# Autodesk Inventor assembly: Assembly1
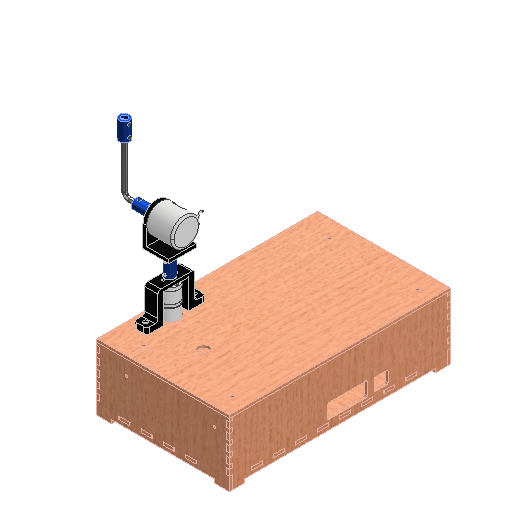
[picture p0: Inventor's stored thumbnail of the model, 512x512]
Saved by Autodesk Inventor 2025.2 (Build 292293000, 293)
## iProperties
Created: 2025-12-07
Part Number: Assembly1
Document SubType Name: Assembly
Designer: hazem
Author: hazem
## Documents named in this file (16)
- D:\Senior 2 MCT\Fall 2025\Hybrid Control\Project\CAD\Workspaces\Workspace\Assembly1.iam
- D:\Senior 2 MCT\Fall 2025\Hybrid Control\Project\CAD\Workspaces\Workspace\Encoder_Default_sldprt.ipt
- D:\Senior 2 MCT\Fall 2025\Hybrid Control\Project\CAD\Workspaces\Workspace\encoderBracketInventor.stp_Default_sldprt.ipt
- D:\Senior 2 MCT\Fall 2025\Hybrid Control\Project\CAD\Workspaces\Workspace\Motor_Default_sldprt.ipt
- D:\Senior 2 MCT\Fall 2025\Hybrid Control\Project\CAD\Workspaces\Workspace\Upper.ipt
- D:\Senior 2 MCT\Fall 2025\Hybrid Control\Project\CAD\Workspaces\Workspace\ground.ipt
- D:\Senior 2 MCT\Fall 2025\Hybrid Control\Project\CAD\Workspaces\Workspace\side.ipt
- D:\Senior 2 MCT\Fall 2025\Hybrid Control\Project\CAD\Workspaces\Workspace\Allen 5 mm.ipt
- D:\Senior 2 MCT\Fall 2025\Hybrid Control\Project\CAD\Workspaces\Workspace\Shaft Coupler 8-5mm.ipt
- D:\Senior 2 MCT\Fall 2025\Hybrid Control\Project\CAD\Workspaces\Workspace\side2.ipt
- D:\Senior 2 MCT\Fall 2025\Hybrid Control\Project\CAD\Workspaces\Workspace\back.ipt
- D:\Senior 2 MCT\Fall 2025\Hybrid Control\Project\CAD\Workspaces\Workspace\Front.ipt
- D:\Senior 2 MCT\Fall 2025\Hybrid Control\Project\CAD\Workspaces\Workspace\L connection.ipt
- D:\Senior 2 MCT\Fall 2025\Hybrid Control\Project\CAD\Workspaces\Workspace\Motor _Fixation.ipt
- D:\Senior 2 MCT\Fall 2025\Hybrid Control\Project\CAD\Workspaces\Workspace\AcoplamentoRigido8x8.ipt
- D:\Senior 2 MCT\Fall 2025\Hybrid Control\Project\CAD\Workspaces\Workspace\Motor Sleeve 0.2.ipt
## Components (22 placed, 15 different names)
1. ground:1 — Mate:31, Flush:12, Flush:13, Mate:39
2. Upper:1 — Flush:7, Flush:9, Flush:10, Mate:46, Mate:49, Mate:50, Mate:53
3. side:1 — Flush:7, Flush:9, Mate:31, Flush:12, Flush:13, Flush:17, Flush:20, Mate:44, Mate:45, Mate:47, Mate:48
4. side2:1 — Flush:10, Flush:18, Flush:21, Mate:51, Mate:52, Mate:54, Mate:55, Flush:22, Mate:56
5. Shaft Coupler 8-5mm:1 — Mate:35, Flush:14
6. Allen 5 mm:1 — Mate:35, Flush:14
7. back:1 — Mate:39, Flush:17, Flush:18, Mate:56, Mate:57
8. Front:1 — Flush:20, Flush:21, Flush:22
9. L connection:1 — Mate:47, Mate:48, Mate:49
10. L connection:2 — Mate:44, Mate:45, Mate:46, Mate:58
11. L connection:3 — Mate:50, Mate:51, Mate:52
12. L connection:4 — Mate:53, Mate:54, Mate:55, Mate:59
13. Motor _Fixation:1 — Mate:61, Mate:62, Mate:63, Mate:64
14. Motor_Default_sldprt:1 — Mate:60, Mate:61, Mate:62, Mate:65, Flush:23
15. Upper:2 — Mate:57, Mate:58, Mate:59, Mate:60, Mate:63, Mate:64
16. AcoplamentoRigido8x8:1 — Mate:66, Flush:24, Mate:67, Mate:68
17. Motor Sleeve 0.2:1 — Mate:65, Flush:23, Mate:66, Flush:24
18. Encoder_Default_sldprt:1 — Mate:69, Mate:70, Mate:71, Mate:72, Mate:75, Mate:76
19. encoderBracketInventor.stp_Default_sldprt:1 — Mate:67, Mate:68, Mate:69, Mate:70, Mate:71, Mate:72
20. Shaft Coupler 8-5mm:2 — Mate:74, Flush:26, Mate:75, Mate:76
21. Shaft Coupler 8-5mm:3 — Mate:73, Flush:25
22. Allen 5 mm:2 — Mate:73, Flush:25, Mate:74, Flush:26
## Relationships (51: Mate 36, Flush 15)
- Flush:7: Upper:1 ↔ side:1
- Flush:9: Upper:1 ↔ side:1
- Flush:10: Upper:1 ↔ side2:1
- Mate:31: ground:1 ↔ side:1
- Flush:12: ground:1 ↔ side:1
- Flush:13: ground:1 ↔ side:1
- Mate:35: Shaft Coupler 8-5mm:1 ↔ Allen 5 mm:1
- Flush:14: Shaft Coupler 8-5mm:1 ↔ Allen 5 mm:1
- Mate:39: ground:1 ↔ back:1
- Flush:17: side:1 ↔ back:1
- Flush:18: side2:1 ↔ back:1
- Flush:20: side:1 ↔ Front:1
- Flush:21: side2:1 ↔ Front:1
- Mate:44: side:1 ↔ L connection:2
- Mate:45: side:1 ↔ L connection:2
- Mate:46: Upper:1 ↔ L connection:2
- Mate:47: side:1 ↔ L connection:1
- Mate:48: side:1 ↔ L connection:1
- Mate:49: Upper:1 ↔ L connection:1
- Mate:50: Upper:1 ↔ L connection:3
- Mate:51: side2:1 ↔ L connection:3
- Mate:52: side2:1 ↔ L connection:3
- Mate:53: Upper:1 ↔ L connection:4
- Mate:54: side2:1 ↔ L connection:4
- Mate:55: side2:1 ↔ L connection:4
- Flush:22: side2:1 ↔ Front:1
- Mate:56: side2:1 ↔ back:1
- Mate:57: back:1 ↔ Upper:2
- Mate:58: L connection:2 ↔ Upper:2
- Mate:59: L connection:4 ↔ Upper:2
- Mate:60: Motor_Default_sldprt:1 ↔ Upper:2
- Mate:61: Motor _Fixation:1 ↔ Motor_Default_sldprt:1
- Mate:62: Motor _Fixation:1 ↔ Motor_Default_sldprt:1
- Mate:63: Motor _Fixation:1 ↔ Upper:2
- Mate:64: Motor _Fixation:1 ↔ Upper:2
- Mate:65: Motor_Default_sldprt:1 ↔ Motor Sleeve 0.2:1
- Flush:23: Motor_Default_sldprt:1 ↔ Motor Sleeve 0.2:1
- Mate:66: AcoplamentoRigido8x8:1 ↔ Motor Sleeve 0.2:1
- Flush:24: AcoplamentoRigido8x8:1 ↔ Motor Sleeve 0.2:1
- Mate:67: AcoplamentoRigido8x8:1 ↔ encoderBracketInventor.stp_Default_sldprt:1
- Mate:68: AcoplamentoRigido8x8:1 ↔ encoderBracketInventor.stp_Default_sldprt:1
- Mate:69: Encoder_Default_sldprt:1 ↔ encoderBracketInventor.stp_Default_sldprt:1
- Mate:70: Encoder_Default_sldprt:1 ↔ encoderBracketInventor.stp_Default_sldprt:1
- Mate:71: Encoder_Default_sldprt:1 ↔ encoderBracketInventor.stp_Default_sldprt:1
- Mate:72: Encoder_Default_sldprt:1 ↔ encoderBracketInventor.stp_Default_sldprt:1
- Mate:73: Shaft Coupler 8-5mm:3 ↔ Allen 5 mm:2
- Flush:25: Shaft Coupler 8-5mm:3 ↔ Allen 5 mm:2
- Mate:74: Shaft Coupler 8-5mm:2 ↔ Allen 5 mm:2
- Flush:26: Shaft Coupler 8-5mm:2 ↔ Allen 5 mm:2
- Mate:75: Encoder_Default_sldprt:1 ↔ Shaft Coupler 8-5mm:2
- Mate:76: Encoder_Default_sldprt:1 ↔ Shaft Coupler 8-5mm:2
## Named parameters: Wood_thickness = 4 mm
